# Autodesk Inventor assembly: Übertragung des Zahnriemens
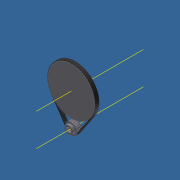
[picture p0: Inventor's stored thumbnail of the model, 180x180]
Saved by Autodesk Inventor 2016 (Build 200138000, 138)
## iProperties
Created: 2015-01-06
Part Number: Übertragung des Zahnriemens
Document SubType Name: Assembly
Designer: 4ndreas
ClientObjectVersion: 1
Author: 4ndreas
## Documents named in this file (6)
- C:\Users\4ndreas\Documents\Inventor\RobotARM v2\v2\BaseJoint\Konstruktions-Assistent\Übertragung des Zahnriemens1.iam
- C:\Users\4ndreas\Documents\Inventor\RobotARM v2\v2\BaseJoint\Konstruktions-Assistent\Zahnriemen1.ipt
- C:\Users\4ndreas\Documents\Inventor\RobotARM v2\v2\BaseJoint\Konstruktions-Assistent\Synchrone Riemenscheibe11.ipt
- C:\Users\4ndreas\Documents\Inventor\RobotARM v2\v2\BaseJoint\Konstruktions-Assistent\Synchrone Riemenscheibe21.ipt
- C:\Users\4ndreas\Documents\Inventor\RobotARM v2\v3\Shoulder\Konstruktions-Assistent\Flache Riemenscheibe11.ipt
- C:\Users\4ndreas\Documents\Inventor\RobotARM v2\v3\Shoulder\Konstruktions-Assistent\Flache Riemenscheibe21.ipt
## Components (5 placed, 5 different names)
1. Zahnriemen:1 — Fluchtend:1, Passend:1, Passend:2, Fluchtend:2, Passend:3, Fluchtend:3, Passend:4, Passend:5, Fluchtend:4, Passend:6
2. Synchrone Riemenscheibe1:1 — Fluchtend:1, Passend:1, Passend:2, Drehung:1, Drehung:2, Drehung:3
3. Synchrone Riemenscheibe2:1 — Fluchtend:3, Passend:4, Drehung:2, Passend:5
4. Flache Riemenscheibe1:1 — Fluchtend:2, Passend:3, Drehung:1
5. Flache Riemenscheibe2:1 — Fluchtend:4, Passend:6, Drehung:3
## Relationships (13: Mate 6, Flush 4, RelateRotation 3)
- Fluchtend:1 [Flush]: Zahnriemen:1 ↔ Synchrone Riemenscheibe1:1
- Passend:1 [Mate]: Zahnriemen:1 ↔ Synchrone Riemenscheibe1:1
- Passend:2 [Mate]: Zahnriemen:1 ↔ Synchrone Riemenscheibe1:1
- Fluchtend:2 [Flush] (-4.5 mm): Zahnriemen:1 ↔ Flache Riemenscheibe1:1
- Passend:3 [Mate]: Zahnriemen:1 ↔ Flache Riemenscheibe1:1
- Drehung:1 [RelateRotation] (0.1303 ul): Synchrone Riemenscheibe1:1 ↔ Flache Riemenscheibe1:1
- Fluchtend:3 [Flush]: Zahnriemen:1 ↔ Synchrone Riemenscheibe2:1
- Passend:4 [Mate]: Zahnriemen:1 ↔ Synchrone Riemenscheibe2:1
- Drehung:2 [RelateRotation] (0.2439 ul): Synchrone Riemenscheibe1:1 ↔ Synchrone Riemenscheibe2:1
- Passend:5 [Mate]: Zahnriemen:1 ↔ Synchrone Riemenscheibe2:1
- Fluchtend:4 [Flush] (-4.5 mm): Zahnriemen:1 ↔ Flache Riemenscheibe2:1
- Passend:6 [Mate]: Zahnriemen:1 ↔ Flache Riemenscheibe2:1
- Drehung:3 [RelateRotation] (0.1073 ul): Synchrone Riemenscheibe1:1 ↔ Flache Riemenscheibe2:1
